# Autodesk Inventor assembly: Nozzle
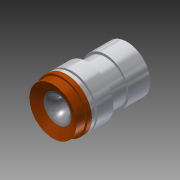
[picture p0: Inventor's stored thumbnail of the model, 180x180]
Saved by Autodesk Inventor 2015 (Build 190159000, 159)
## iProperties
Created: 2016-01-09
Part Number: Nozzle
Document SubType Name: Assembly
Designer: Jared
Author: Jared
## Documents named in this file (6)
- D:\Google Drive\TRC Members\3. IPT (Integrated Product Teams)\Propulsion\2015-2016 Year\6 in Motor\CAD\Flight Motor\Version 3\Nozzle.iam
- D:\Google Drive\TRC Members\3. IPT (Integrated Product Teams)\Propulsion\2015-2016 Year\6 in Motor\CAD\Flight Motor\Version 3\Nozzle\Aluminum Carrier.ipt
- D:\Google Drive\TRC Members\3. IPT (Integrated Product Teams)\Propulsion\2015-2016 Year\6 in Motor\CAD\Flight Motor\Version 3\Nozzle\Aluminum Retainer.ipt
- D:\Google Drive\TRC Members\3. IPT (Integrated Product Teams)\Propulsion\2015-2016 Year\6 in Motor\CAD\Flight Motor\Version 3\Nozzle\Aluminum Skirt.ipt
- D:\Google Drive\TRC Members\3. IPT (Integrated Product Teams)\Propulsion\2015-2016 Year\6 in Motor\CAD\Flight Motor\Version 3\Nozzle\Graphite.ipt
- D:\Google Drive\TRC Members\3. IPT (Integrated Product Teams)\Propulsion\2015-2016 Year\6 in Motor\CAD\Flight Motor\Version 3\Nozzle\Phenolic.ipt
## Components (5 placed, 5 different names)
1. Aluminum Carrier:1 — Mate:2, Mate:4, Mate:6, Mate:7, Mate:8
2. Aluminum Retainer:1 — Mate:3, Mate:7
3. Aluminum Skirt:1 — Mate:4, Mate:8, Mate:9, Mate:10
4. Graphite:1 — Mate:1, Mate:5
5. Phenolic:1 — Mate:1, Mate:2, Mate:3, Mate:5, Mate:6
## Relationships (10: Mate 10)
- Mate:1: Graphite:1 ↔ Phenolic:1
- Mate:2: Aluminum Carrier:1 ↔ Phenolic:1
- Mate:3: Aluminum Retainer:1 ↔ Phenolic:1
- Mate:4: Aluminum Carrier:1 ↔ Aluminum Skirt:1
- Mate:5: Graphite:1 ↔ Phenolic:1
- Mate:6: Aluminum Carrier:1 ↔ Phenolic:1
- Mate:7: Aluminum Carrier:1 ↔ Aluminum Retainer:1
- Mate:8: Aluminum Carrier:1 ↔ Aluminum Skirt:1
- Mate:9: Aluminum Skirt:1
- Mate:10: Aluminum Skirt:1
